# Autodesk Inventor assembly: sb_assembly
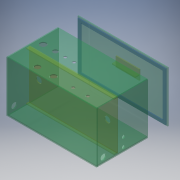
[picture p0: Inventor's stored thumbnail of the model, 180x180]
Saved by Autodesk Inventor 2018.1 (Build 221171000, 171)
## iProperties
Created: 2017-08-17
Part Number: sb_assembly
Document SubType Name: Assembly
Designer: Tom
Author: Tom
## Documents named in this file (9)
- \\Mac\Dropbox\2015-2016\Bachelorproef\Inventor\Electronics and Solenoids Box\eb_assembly.iam
- \\Mac\Dropbox\2015-2016\Bachelorproef\Inventor\Electronics and Solenoids Box\eb_bottom.ipt
- \\Mac\Dropbox\2015-2016\Bachelorproef\Inventor\Electronics and Solenoids Box\eb_front.ipt
- \\Mac\Dropbox\2015-2016\Bachelorproef\Inventor\Electronics and Solenoids Box\eb_left.ipt
- \\Mac\Dropbox\2015-2016\Bachelorproef\Inventor\Electronics and Solenoids Box\eb_lid_assembly.iam
- \\Mac\Dropbox\2015-2016\Bachelorproef\Inventor\Electronics and Solenoids Box\eb_separator_assembly.iam
- \\Mac\Dropbox\2015-2016\Bachelorproef\Inventor\Electronics and Solenoids Box\eb_back.ipt
- \\Mac\Dropbox\2015-2016\Bachelorproef\Inventor\Electronics and Solenoids Box\eb_right.ipt
- \\Mac\Dropbox\2015-2016\Bachelorproef\Inventor\Electronics and Solenoids Box\par_sol_box.xls
## Components (7 placed, 7 different names)
1. eb_bottom:1 — Mate:2, Flush:1, Flush:2, Mate:8, Mate:9, Flush:11, Mate:11, Mate:13
2. eb_front:1 — Mate:2, Flush:1, Flush:2, Flush:10, Mate:6, Flush:12, Flush:13, Flush:16, Mate:16, Mate:17
3. eb_lid_assembly:1 [sub-assembly] — Flush:10, Flush:14, Flush:15, Mate:15, Flush:17
4. eb_separator_assembly:1 [sub-assembly] — Mate:6, Mate:8
5. eb_back:1 — Mate:9, Flush:11, Flush:14, Flush:15, Flush:16
6. eb_left:2 — Mate:11, Flush:12, Mate:17, Flush:17
7. eb_right:1 — Mate:13, Flush:13, Mate:15, Mate:16
## Relationships (19: Flush 10, Mate 9)
- Mate:2: eb_bottom:1 ↔ eb_front:1
- Flush:1: eb_bottom:1 ↔ eb_front:1
- Flush:2 (5 mm): eb_bottom:1 ↔ eb_front:1
- Flush:10: eb_front:1 ↔ eb_lid_assembly:1
- Mate:6: eb_front:1 ↔ eb_separator_assembly:1
- Mate:8 (105 mm): eb_bottom:1 ↔ eb_separator_assembly:1
- Mate:9: eb_bottom:1 ↔ eb_back:1
- Flush:11: eb_bottom:1 ↔ eb_back:1
- Mate:11: eb_bottom:1 ↔ eb_left:2
- Flush:12: eb_front:1 ↔ eb_left:2
- Mate:13: eb_bottom:1 ↔ eb_right:1
- Flush:13: eb_front:1 ↔ eb_right:1
- Flush:14: eb_lid_assembly:1 ↔ eb_back:1
- Flush:15: eb_lid_assembly:1 ↔ eb_back:1
- Mate:15: eb_lid_assembly:1 ↔ eb_right:1
- Flush:16: eb_front:1 ↔ eb_back:1
- Mate:16: eb_front:1 ↔ eb_right:1
- Mate:17: eb_front:1 ↔ eb_left:2
- Flush:17: eb_lid_assembly:1 ↔ eb_left:2
## Named parameters: solhole = 3 mm, solholespacing = 16 mm, ssoll = 70 mm, ssolw = 63 mm, bsoll = 126 mm, bsolw = 91 mm, bsolh = 126 mm, tapl = 31 mm, tl = 32 mm, tw = 50 mm, eloboww = 25 mm, pvct = 5 mm, boxw = 450 mm, boxl = 250 mm, boxh = 258 mm, supporth = 15 mm, play = 0.5 mm, sidedist = 90 mm, psul = 140 mm, arl = 102 mm, psuh = 85 mm, screent = 50 mm, screenl = 115 mm, psuw = 150 mm, screenw = 197 mm, pcbw = 76 mm, pcbh = 46 mm, arw = 54 mm, pcbl = 86 mm, seph = 105 mm, dialoadouter = 25 mm, diapowerouter = 25 mm, diaph = 32 mm, distpumps = 75 mm, diaphouter = 48 mm, distbubblewater = 82 mm, diaload = 16 mm, distsidepump = 120 mm, diapower = 16 mm, distpumpbubble = 100 mm, diaetape = 25 mm, diaetapeouter = 36 mm, pumpinner = 16 mm, pumpouter = 25 mm, airoutinner = 28 mm, airininner = 28 mm, waterouter = 39 mm, airoutouter = 39 mm, airinouter = 39 mm, waterinner = 28 mm, distsidewater = 100 mm
